# Autodesk Inventor assembly: Fox_Plus_Robinson
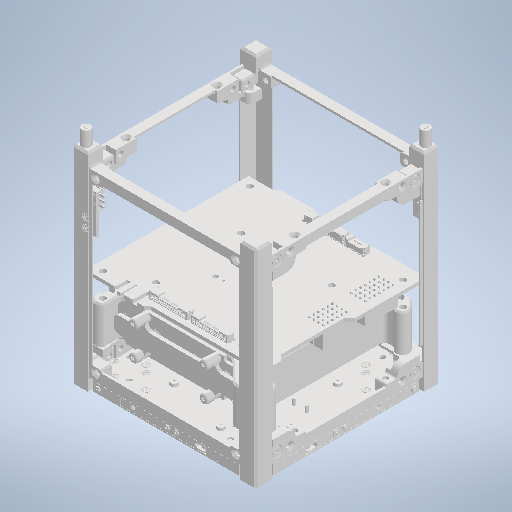
[picture p0: Inventor's stored thumbnail of the model, 512x512]
Saved by Autodesk Inventor 2025 (Build 290162000, 162)
## iProperties
Created: 2024-03-31
Part Number: Fox_Plus_Robinson
Document SubType Name: Assembly
Designer: arobi
Engineer: GAR
Author: Andrew Robinson
Title: Fox Plus Assembly
## Documents named in this file (5)
- C:\Users\arobi\Documents\Repos\fox-plus\mechanical\AssemblyModels\Fox_Plus_AssemblyModel.iam
- C:\Users\arobi\Documents\Repos\fox-plus\mechanical\AssemblyModels\ISIS CubeSat STS PC104 Skeleton.iam
- C:\Users\arobi\Documents\Repos\fox-plus\mechanical\AssemblyModels\ISIS_ANTS1_REVD_STEP_STOWED_asm.iam
- C:\Users\arobi\Documents\Repos\fox-plus\mechanical\AssemblyModels\isis-ipbp4c-3-0-001.ipt
- C:\Users\arobi\Documents\Repos\fox-plus\mechanical\AssemblyModels\isispace-icepsv2-e-1_typeb.ipt
## Components (4 placed, 4 different names)
1. ISIS CubeSat STS PC104 Skeleton:1 [sub-assembly] — Mate:4, Flush:2, Flush:1, Mate:1, Mate:2, Mate:3, Mate:7, Mate:8, Mate:9, Mate:10, Mate:11
2. ISIS_ANTS1_REVD_STEP_STOWED_asm:1 [sub-assembly] — Mate:1, Mate:2, Mate:3
3. isis-ipbp4c-3-0-001:1 — Mate:9, Mate:10, Mate:11, Mate:6
4. isispace-icepsv2-e-1_typeb:1 — Mate:6, Mate:7, Mate:8
## Relationships (12: Mate 10, Flush 2)
- Mate:4: ISIS CubeSat STS PC104 Skeleton:1
- Flush:2: ISIS CubeSat STS PC104 Skeleton:1
- Flush:1: ISIS CubeSat STS PC104 Skeleton:1
- Mate:1: ISIS CubeSat STS PC104 Skeleton:1 ↔ ISIS_ANTS1_REVD_STEP_STOWED_asm:1
- Mate:2: ISIS CubeSat STS PC104 Skeleton:1 ↔ ISIS_ANTS1_REVD_STEP_STOWED_asm:1
- Mate:3: ISIS CubeSat STS PC104 Skeleton:1 ↔ ISIS_ANTS1_REVD_STEP_STOWED_asm:1
- Mate:6 (11 mm): isis-ipbp4c-3-0-001:1 ↔ isispace-icepsv2-e-1_typeb:1
- Mate:7: ISIS CubeSat STS PC104 Skeleton:1 ↔ isispace-icepsv2-e-1_typeb:1
- Mate:8: ISIS CubeSat STS PC104 Skeleton:1 ↔ isispace-icepsv2-e-1_typeb:1
- Mate:9: ISIS CubeSat STS PC104 Skeleton:1 ↔ isis-ipbp4c-3-0-001:1
- Mate:10: ISIS CubeSat STS PC104 Skeleton:1 ↔ isis-ipbp4c-3-0-001:1
- Mate:11: ISIS CubeSat STS PC104 Skeleton:1 ↔ isis-ipbp4c-3-0-001:1
